# Autodesk Inventor assembly: Butterfly Drive Base
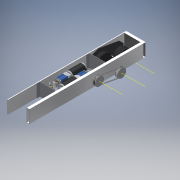
[picture p0: Inventor's stored thumbnail of the model, 180x180]
Saved by Autodesk Inventor 2019.4 (Build 234330000, 330)
## iProperties
Created: 2019-10-19
Part Number: Butterfly Drive Base
Document SubType Name: Assembly
Designer: Mark
Author: Mark
## Documents named in this file (13)
- C:\Users\admin\Desktop\FRC 2020 Engineering\GitHub\7738-CAD-prep\Butterfly drive\Butterfly Drive Base.iam
- C:\Users\admin\Desktop\FRC 2020 Engineering\GitHub\7738-CAD-prep\Butterfly drive\Butterfly Drive Module.iam
- C:\Users\admin\Desktop\FRC 2020 Engineering\GitHub\7738-CAD-prep\Butterfly drive\Side Extrusion.ipt
- C:\Users\admin\Desktop\FRC 2020 Engineering\GitHub\7738-CAD-prep\Butterfly drive\Module Plate 1.ipt
- C:\Users\admin\Desktop\FRC 2020 Engineering\GitHub\7738-CAD-prep\Butterfly drive\Back Extrusion 1.ipt
- C:\Users\admin\Desktop\FRC 2020 Engineering\GitHub\7738-CAD-prep\Butterfly drive\Bumper Plate.ipt
- C:\Users\admin\Desktop\FRC 2020 Engineering\GitHub\7738-CAD-prep\Butterfly drive\Side Front Extrusion.ipt
- C:\Users\admin\Desktop\FRC 2020 Engineering\GitHub\7738-CAD-prep\Butterfly drive\F6800Z 10mm ID Flange.ipt
- C:\Users\admin\Desktop\FRC 2020 Engineering\GitHub\7738-CAD-prep\Butterfly drive\Butterfly Drive Base\Design Accelerator\Synchronous Belts Transmission1.iam
- C:\Users\admin\Desktop\FRC 2020 Engineering\GitHub\7738-CAD-prep\2 Stage HD - CIM Sport.iam
- C:\Users\admin\Desktop\FRC 2020 Engineering\GitHub\7738-CAD-prep\am-0255 2.5inch CIM Motor.ipt
- C:\Users\admin\Desktop\FRC 2020 Engineering\GitHub\7738-CAD-prep\Butterfly drive\Spacer Extrusion.ipt
- C:\Users\admin\Desktop\FRC 2020 Engineering\GitHub\7738-CAD-prep\Butterfly drive\Butterfly Drive Base\Design Accelerator\Bevel Gears2.iam
## Components (16 placed, 11 different names)
1. Butterfly Drive Module:1 [sub-assembly] — Angle:1, Mate:8, Mate:11, Mate:13, Mate:28
2. Side Extrusion:1 — Mate:1, Flush:1, Angle:1, Flush:7, Mate:10, Flush:8, Mate:12, Mate:14, Flush:9, Mate:20, Mate:26, Symmetry:1, Flush:10, Mate:29, Flush:11
3. Back Extrusion 1:1 — Mate:1, Flush:1, Mate:6, Flush:4, Flush:5, Mate:7, Flush:6
4. Bumper Plate:1 — Flush:5, Mate:7, Mate:8, Flush:6, Mate:24, Mate:26, Mate:28, Mate:31
5. Side Front Extrusion:1 — Flush:7, Mate:10, Flush:8, Symmetry:1, Mate:30
6. F6800Z 10mm ID Flange:1 — Mate:11, Mate:12
7. F6800Z 10mm ID Flange:2 — Mate:13, Mate:14
8. Synchronous Belts Transmission:1 [sub-assembly]
9. 2 Stage HD - CIM Sport:1 [sub-assembly] — Mate:15, Mate:16, Mate:17, Mate:20, Mate:33
10. am-0255 2.5inch CIM Motor:1 — Mate:15, Mate:16, Mate:17, Mate:25
11. 2 Stage HD - CIM Sport:2 [sub-assembly] — Mate:24, Mate:32
12. am-0255 2.5inch CIM Motor:2 — Mate:25
13. Spacer Extrusion:2 — Flush:10, Mate:29, Mate:30
14. Spacer Extrusion:3 — Flush:11, Mate:31
15. Bevel Gears:2 [sub-assembly] — Mate:33
16. Bevel Gears:3 [sub-assembly] — Mate:32
## Relationships (36: Mate 25, Flush 9, Angle 1, Symmetry 1)
- Mate:1: Side Extrusion:1 ↔ Back Extrusion 1:1
- Flush:1: Side Extrusion:1 ↔ Back Extrusion 1:1
- Mate:6: Back Extrusion 1:1
- Flush:4: Back Extrusion 1:1
- Angle:1 (10 deg): Butterfly Drive Module:1 ↔ Side Extrusion:1
- Flush:5: Back Extrusion 1:1 ↔ Bumper Plate:1
- Mate:7: Back Extrusion 1:1 ↔ Bumper Plate:1
- Mate:8: Butterfly Drive Module:1 ↔ Bumper Plate:1
- Flush:6: Back Extrusion 1:1 ↔ Bumper Plate:1
- Flush:7: Side Extrusion:1 ↔ Side Front Extrusion:1
- Mate:10: Side Extrusion:1 ↔ Side Front Extrusion:1
- Flush:8: Side Extrusion:1 ↔ Side Front Extrusion:1
- Mate:11: Butterfly Drive Module:1 ↔ F6800Z 10mm ID Flange:1
- Mate:12 (0.3 mm): Side Extrusion:1 ↔ F6800Z 10mm ID Flange:1
- Mate:13: Butterfly Drive Module:1 ↔ F6800Z 10mm ID Flange:2
- Mate:14 (0.3 mm): Side Extrusion:1 ↔ F6800Z 10mm ID Flange:2
- Flush:9 (-18.548 mm): Side Extrusion:1
- Mate:15: 2 Stage HD - CIM Sport:1 ↔ am-0255 2.5inch CIM Motor:1
- Mate:16: 2 Stage HD - CIM Sport:1 ↔ am-0255 2.5inch CIM Motor:1
- Mate:17 (0.6 mm): 2 Stage HD - CIM Sport:1 ↔ am-0255 2.5inch CIM Motor:1
- Mate:20 (10 mm): Side Extrusion:1 ↔ 2 Stage HD - CIM Sport:1
- [Mate]: 2 Stage HD - CIM Sport:2 ↔ am-0255 2.5inch CIM Motor:2
- [Mate]: 2 Stage HD - CIM Sport:2 ↔ am-0255 2.5inch CIM Motor:2
- [Mate] (0.6 mm): 2 Stage HD - CIM Sport:2 ↔ am-0255 2.5inch CIM Motor:2
- Mate:24 (10 mm): Bumper Plate:1 ↔ 2 Stage HD - CIM Sport:2
- Mate:25 (1.5 mm): am-0255 2.5inch CIM Motor:1 ↔ am-0255 2.5inch CIM Motor:2
- Mate:26 (126 mm): Side Extrusion:1 ↔ Bumper Plate:1
- Symmetry:1: Side Extrusion:1 ↔ Side Front Extrusion:1
- Mate:28 (0.3 mm): Butterfly Drive Module:1 ↔ Bumper Plate:1
- Flush:10: Side Extrusion:1 ↔ Spacer Extrusion:2
- Mate:29: Side Extrusion:1 ↔ Spacer Extrusion:2
- Mate:30 (270 mm): Side Front Extrusion:1 ↔ Spacer Extrusion:2
- Flush:11: Side Extrusion:1 ↔ Spacer Extrusion:3
- Mate:31 (0.5 mm): Bumper Plate:1 ↔ Spacer Extrusion:3
- Mate:32: 2 Stage HD - CIM Sport:2 ↔ Bevel Gears:3
- Mate:33: 2 Stage HD - CIM Sport:1 ↔ Bevel Gears:2
## Named parameters: Height = 80 mm, ExtSta = 1 deg, ModuleAngle = 10 deg, d58_d50 = 0.6 mm, d59_d48 = 0 mm, d60_d49 = 0 mm
